# Autodesk Inventor assembly: teljes3
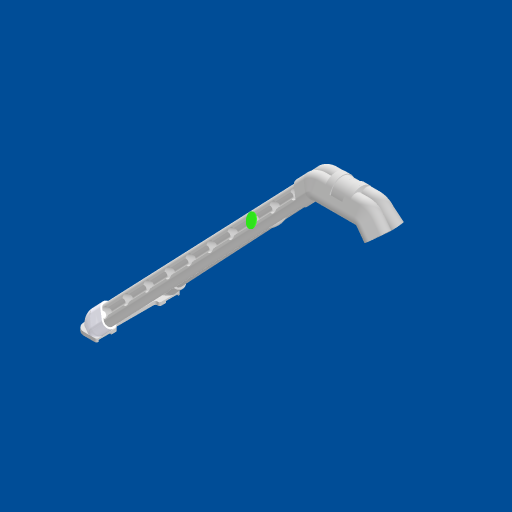
[picture p0: Inventor's stored thumbnail of the model, 512x512]
Saved by Autodesk Inventor 2023 (Build 270158000, 158)
## iProperties
Created: 2022-11-11
Part Number: teljes3
Document SubType Name: Assembly
Designer: gd1
Author: gd1
## Documents named in this file (6)
- C:\Users\gd1\3D Objects\3D nagyteherbírású híd\Híd\H-d\teljes7.iam
- C:\Users\gd1\3D Objects\3D nagyteherbírású híd\Híd\H-d\palca 325mm.ipt
- C:\Users\gd1\3D Objects\3D nagyteherbírású híd\Híd\H-d\tipli.ipt
- C:\Users\gd1\3D Objects\3D nagyteherbírású híd\Híd\H-d\kozepcsati2.iam
- C:\Users\gd1\3D Objects\3D nagyteherbírású híd\Híd\H-d\45 fok középre_talp másolata.ipt
- C:\Users\gd1\3D Objects\3D nagyteherbírású híd\Híd\H-d\osszekotoelem.iam
## Components (9 placed, 5 different names)
1. palca 325mm:1 — Rotational:5, Rotational:6
2. palca 325mm:2 — Rotational:4
3. tipli:1
4. tipli:2
5. kozepcsati2:1 [sub-assembly] — Rotational:4
6. 45 fok középre_talp másolata:1 — Rotational:5
7. osszekotoelem:1 [sub-assembly] — Rotational:6, Rotational:7, Rotational:8
8. tipli:3 — Rotational:7
9. tipli:4 — Rotational:8
## Relationships (5: RevoluteJoint 5)
- Rotational:4 [RevoluteJoint]: palca 325mm:2 ↔ kozepcsati2:1
- Rotational:5 [RevoluteJoint]: palca 325mm:1 ↔ 45 fok középre_talp másolata:1
- Rotational:6 [RevoluteJoint]: palca 325mm:1 ↔ osszekotoelem:1
- Rotational:7 [RevoluteJoint]: osszekotoelem:1 ↔ tipli:3
- Rotational:8 [RevoluteJoint]: osszekotoelem:1 ↔ tipli:4
